# Autodesk Inventor assembly: Rod End 8mm
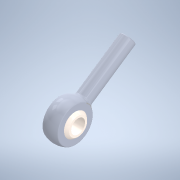
[picture p0: Inventor's stored thumbnail of the model, 180x180]
Saved by Autodesk Inventor 2021 (Build 250183000, 183)
## iProperties
Created: 2022-09-08
Part Number: Rod End 8mm
Document SubType Name: Assembly
Designer: Administrator
Title: Rod End 8mm P v1
Author: Administrator
## Documents named in this file (3)
- C:\Users\szucs\Desktop\GTPR\ver2\Rod End 8mm.iam
- C:\Users\szucs\Desktop\GTPR\ver2\outer.ipt
- C:\Users\szucs\Desktop\GTPR\ver2\inner.ipt
## Components (2 placed, 2 different names)
1. outer:1 — Tangent:1
2. inner:1 — Tangent:1
## Relationships (1: Tangent 1)
- Tangent:1: outer:1 ↔ inner:1
